# Autodesk Inventor assembly: torsosc-support
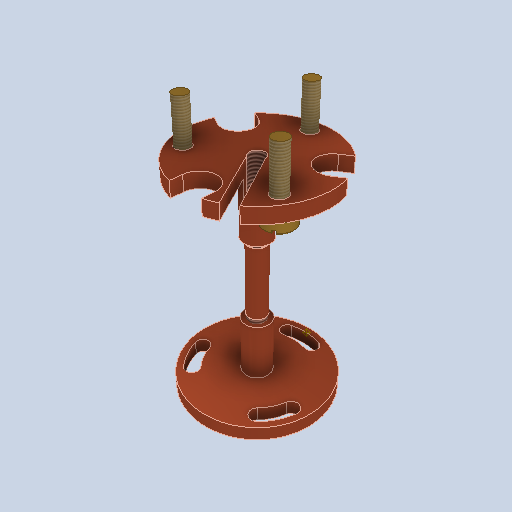
[picture p0: Inventor's stored thumbnail of the model, 512x512]
Saved by Autodesk Inventor 2026 (Build 300175050, 175E)
## iProperties
Created: 2026-02-13
Part Number: torsosc-support
Document SubType Name: Assembly
Designer: schanen
Author: schanen
## Documents named in this file (5)
- C:\Users\schanen\Documents\work-experiments-torsosc-2026\inventor\torsosc-support.iam
- C:\Users\schanen\Documents\work-experiments-torsosc-2026\inventor\torsosc-support-flange-bottom.ipt
- C:\Users\schanen\Documents\work-experiments-torsosc-2026\inventor\torsosc-support-flange-top.ipt
- C:\Users\schanen\Documents\work-experiments-torsosc-2026\inventor\torsosc-support-link.ipt
- C:\Users\schanen\Documents\work-experiments-torsosc-2026\inventor\Screw-CheeseHead-Brass-M3x12.ipt
## Components (6 placed, 4 different names)
1. torsosc-support-flange-bottom:1 — Mate:2, Mate:4, Mate:6, Mate:8, Mate:9
2. torsosc-support-flange-top:1 — Mate:1, Mate:3, Mate:7
3. torsosc-support-link:1 — Mate:1, Mate:2, Mate:3, Mate:4, Mate:5
4. Screw-CheeseHead-Brass-M3x12:1 — Mate:8, Mate:9
5. Screw-CheeseHead-Brass-M3x12:2
6. Screw-CheeseHead-Brass-M3x12:3
## Component patterns: (3 elements, first: Screw-CheeseHead-Brass-M3x12:1)
## Relationships (9: Mate 9)
- Mate:1: torsosc-support-flange-top:1 ↔ torsosc-support-link:1
- Mate:2: torsosc-support-flange-bottom:1 ↔ torsosc-support-link:1
- Mate:3 (-4 mm): torsosc-support-flange-top:1 ↔ torsosc-support-link:1
- Mate:4 (-4 mm): torsosc-support-flange-bottom:1 ↔ torsosc-support-link:1
- Mate:5: torsosc-support-link:1
- Mate:6: torsosc-support-flange-bottom:1
- Mate:7: torsosc-support-flange-top:1
- Mate:8: torsosc-support-flange-bottom:1 ↔ Screw-CheeseHead-Brass-M3x12:1
- Mate:9: torsosc-support-flange-bottom:1 ↔ Screw-CheeseHead-Brass-M3x12:1
